# Autodesk Inventor assembly: vwheel
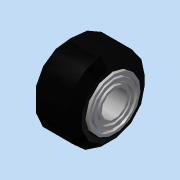
[picture p0: Inventor's stored thumbnail of the model, 180x180]
Saved by Autodesk Inventor 2015 (Build 190159000, 159)
## iProperties
Created: 2016-09-08
Part Number: vwheel
Document SubType Name: Assembly
Designer: Dustin
Author: Dustin
## Documents named in this file (3)
- E:\Documents\3D Printer\Parts\New Printer\vwheel.iam
- E:\Documents\3D Printer\Parts\New Printer\V Slot Part Files\Pulleys Wheels Bearings\Mini Bearing.ipt
- E:\Documents\3D Printer\Parts\New Printer\V Slot Part Files\Pulleys Wheels Bearings\Micro V Wheel.ipt
## Components (3 placed, 2 different names)
1. Mini Bearing:1 — Insert:2
2. Mini Bearing:2 — Insert:1
3. Micro V Wheel:1 — Insert:1, Insert:2
## Relationships (2: Insert 2)
- Insert:1: Mini Bearing:2 ↔ Micro V Wheel:1
- Insert:2: Mini Bearing:1 ↔ Micro V Wheel:1
